# Autodesk Inventor assembly: Red Pump Pipe H w_ sensors v1
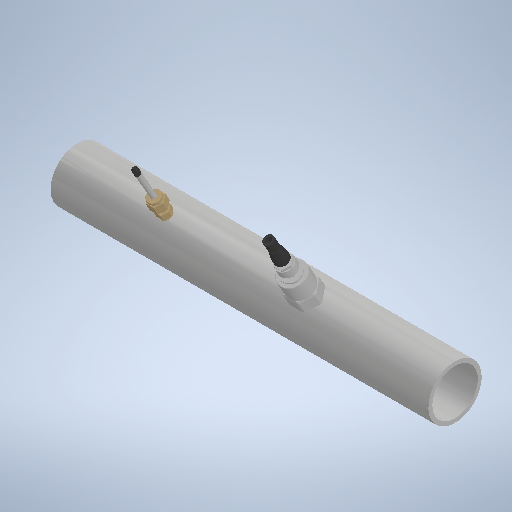
[picture p0: Inventor's stored thumbnail of the model, 512x512]
Saved by Autodesk Inventor 2027 (Build 310192000, 192)
## iProperties
Created: 2026-07-30
Part Number: Red Pump Pipe H w_ sensors v1
Document SubType Name: Assembly
Designer: AdminForWorker
Title: Pipe H w/ sensors v1
Author: AdminForWorker
## Documents named in this file (4)
- C:\Users\ig2\Desktop\Inventor stuff on your own\Red Pump Pipe H w_ sensors v1.iam
- C:\Users\ig2\Desktop\Inventor stuff on your own\Red Pump Pipe H v4.ipt
- C:\Users\ig2\Desktop\Inventor stuff on your own\Red Pump 0-60 PSI Transducer v2.ipt
- C:\Users\ig2\Desktop\Inventor stuff on your own\Red Pump New Thermal Couple Complete v2_2.iam
## Components (3 placed, 3 different names)
1. Red Pump Pipe H v4:1 — Rigid:1, Rigid:2
2. Red Pump 0-60 PSI Transducer v2:1 — Rigid:2
3. Red Pump New Thermal Couple Complete v2_2:1 [sub-assembly] — Rigid:1
## Relationships (2: WeldJoint 2)
- Rigid:1 [WeldJoint] (-6.35 mm): Red Pump Pipe H v4:1 ↔ Red Pump New Thermal Couple Complete v2_2:1
- Rigid:2 [WeldJoint]: Red Pump Pipe H v4:1 ↔ Red Pump 0-60 PSI Transducer v2:1
